# Autodesk Inventor assembly: Drone
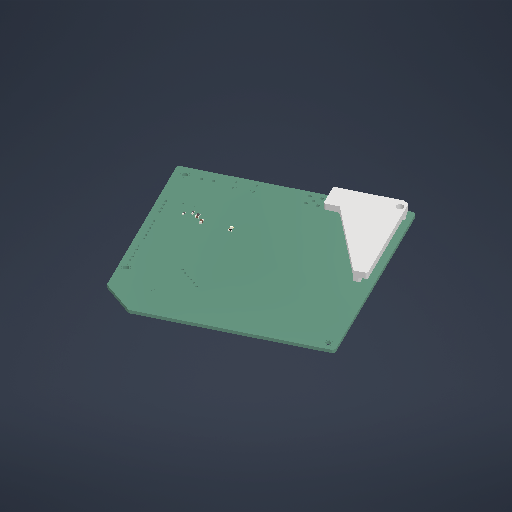
[picture p0: Inventor's stored thumbnail of the model, 512x512]
Saved by Autodesk Inventor 2026.1 (Build 301233020, 233B)
## iProperties
Created: 2026-04-22
Part Number: Drone
Document SubType Name: Assembly
Designer: Mikke
Author: Mikke
## Documents named in this file (4)
- C:\Users\Mikke\OneDrive - Aalborg Universitet\ESD 610 - General\Inventor\Drone_build\Drone.iam
- C:\Users\Mikke\OneDrive - Aalborg Universitet\ESD 610 - General\Inventor\Drone_build\Bund.ipt
- C:\Users\Mikke\OneDrive - Aalborg Universitet\ESD 610 - General\Inventor\Drone_build\Board\Board\Board.iam
- C:\Users\Mikke\OneDrive - Aalborg Universitet\ESD 610 - General\Inventor\Drone_build\SnapHolder.ipt
## Components (3 placed, 3 different names)
1. Bund:1 — Mate:1
2. Board:1 [sub-assembly] — Mate:1, Flush:1, Flush:2
3. SnapHolder:1 — Flush:1, Flush:2
## Relationships (3: Flush 2, Mate 1)
- Mate:1: Bund:1 ↔ Board:1
- Flush:1: Board:1 ↔ SnapHolder:1
- Flush:2: Board:1 ↔ SnapHolder:1
